# Autodesk Inventor assembly: PreFinal
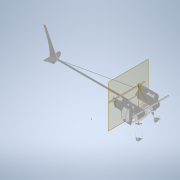
[picture p0: Inventor's stored thumbnail of the model, 180x180]
Saved by Autodesk Inventor 2020 (Build 240168000, 168)
## iProperties
Created: 2019-06-03
Part Number: PreFinal
Document SubType Name: Assembly
Designer: Vivek Muskan
Author: Vivek Muskan
## Documents named in this file (9)
- C:\Users\Vivek Muskan\Documents\TARGET25\PreFinal.iam
- C:\Users\Vivek Muskan\Documents\TARGET25\PreFinal\Design Accelerator\Bevel Gears2.iam
- C:\Users\Vivek Muskan\Documents\TARGET25\sharft.ipt
- C:\Users\Vivek Muskan\Documents\TARGET25\SwashBase.ipt
- C:\Users\Vivek Muskan\Documents\TARGET25\SwashBobble.ipt
- C:\Users\Vivek Muskan\Documents\TARGET25\SwashTop.ipt
- C:\Users\Vivek Muskan\Documents\TARGET25\OneWayBearing.ipt
- C:\Users\Vivek Muskan\Documents\TARGET25\PreFinal\Design Accelerator\Spur Gears5.iam
- C:\Users\Vivek Muskan\Documents\TARGET25\syncFrame.iam
## Components (12 placed, 8 different names)
1. Bevel Gears:1 [sub-assembly] — Insert:1, Mate:6, Flush:1, Flush:2, Mate:11
2. OneWayBearing:1 — Mate:1, Mate:2
3. sharft:1 — Mate:3, Mate:5, Mate:6, Flush:1
4. sharft:2 — Mate:7, Mate:8, Mate:10, Flush:2, Mate:11
5. SwashBase:1 — Mate:4, Mate:5
6. SwashBobble:1 — Mate:3, Insert:2
7. SwashTop:1 — Insert:2, Mate:4
8. SwashBase:2 — Mate:9, Mate:10
9. SwashBobble:2 — Mate:7, Insert:3
10. SwashTop:2 — Mate:8, Insert:3, Mate:9
11. Spur Gears:1 [sub-assembly] — Mate:1, Mate:2, Insert:1
12. syncFrame:1 [sub-assembly] — Flush:3, Flush:4, Flush:5
## Relationships (19: Mate 11, Flush 5, Insert 3)
- Mate:1: OneWayBearing:1 ↔ Spur Gears:1
- Mate:2: OneWayBearing:1 ↔ Spur Gears:1
- Insert:1 (3 mm): Bevel Gears:1 ↔ Spur Gears:1
- Mate:3: sharft:1 ↔ SwashBobble:1
- Insert:2 (8 mm): SwashBobble:1 ↔ SwashTop:1
- Mate:4: SwashBase:1 ↔ SwashTop:1
- Mate:5: sharft:1 ↔ SwashBase:1
- Mate:6: Bevel Gears:1 ↔ sharft:1
- Flush:1: Bevel Gears:1 ↔ sharft:1
- Mate:7: sharft:2 ↔ SwashBobble:2
- Mate:8: sharft:2 ↔ SwashTop:2
- Insert:3 (8 mm): SwashBobble:2 ↔ SwashTop:2
- Mate:9: SwashBase:2 ↔ SwashTop:2
- Mate:10: sharft:2 ↔ SwashBase:2
- Flush:2: Bevel Gears:1 ↔ sharft:2
- Mate:11: Bevel Gears:1 ↔ sharft:2
- Flush:3 (140 mm): syncFrame:1
- Flush:4 (-420 mm): syncFrame:1
- Flush:5: syncFrame:1
